# Autodesk Inventor assembly: 093_CPY
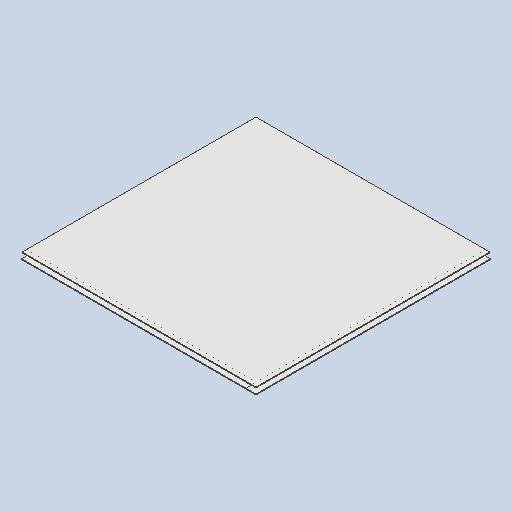
[picture p0: Inventor's stored thumbnail of the model, 512x512]
Saved by Autodesk Inventor 2026.2 (Build 302298000, 298)
## iProperties
Created: 2026-05-19
Part Number: 093_CPY
Document SubType Name: Assembly
Designer: user
Author: user
## Documents named in this file (4)
- C:\Users\admin\Documents\Inventor\GBK-Gubkinskiy\093_CPY.iam
- C:\Users\admin\Documents\Inventor\GBK-Gubkinskiy\0931_CPY.ipt
- C:\Users\admin\Documents\Inventor\GBK-Gubkinskiy\0932_CPY.ipt
- C:\Users\admin\Documents\Inventor\GBK-Gubkinskiy\0933_CPY.ipt
## Components (3 placed, 3 different names)
1. 0931_CPY:1 — Flush:1, Mate:1, Flush:2
2. 0932_CPY:1 — Flush:1, Mate:1, Rigid:1
3. 0933_CPY:1 — Flush:2, Rigid:1
## Relationships (4: Flush 2, Mate 1, WeldJoint 1)
- Flush:1 (34 mm): 0931_CPY:1 ↔ 0932_CPY:1
- Mate:1: 0931_CPY:1 ↔ 0932_CPY:1
- Flush:2 (34 mm): 0931_CPY:1 ↔ 0933_CPY:1
- Rigid:1 [WeldJoint]: 0932_CPY:1 ↔ 0933_CPY:1
